# Autodesk Inventor assembly: ensamble
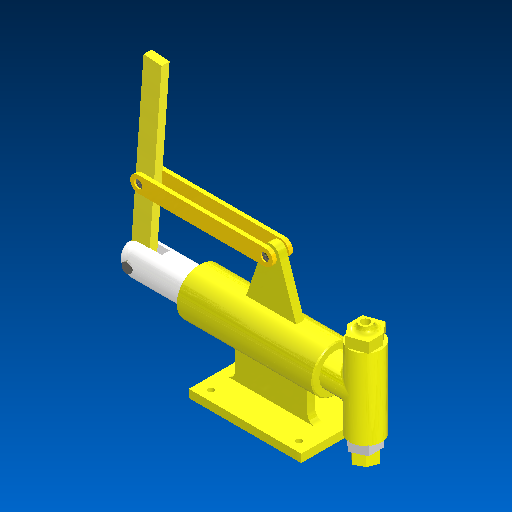
[picture p0: Inventor's stored thumbnail of the model, 512x512]
Saved by Autodesk Inventor 2025.2 (Build 292293000, 293)
## iProperties
Created: 2024-11-13
Part Number: ensamble
Document SubType Name: Assembly
Designer: Steven C
Author: Steven C
## Documents named in this file (12)
- C:\Users\Steven C\Desktop\8-807\ensamble.iam
- C:\Users\Steven C\Desktop\8-807\1 HUDSON-8-28A-TDR HAND PUMP BASE BODY.ipt
- C:\Users\Steven C\Desktop\8-807\1 -HUDSON-8-31B-TDR HAND PUMP PISTON.ipt
- C:\Users\Steven C\Desktop\8-807\1-HUDSON-8-29-TDR HAND PUMP BODY TOP OUTLET.ipt
- C:\Users\Steven C\Desktop\8-807\1-HUDSON-8-30-TDR HAND PUMP BODY BOTTOM INLET.ipt
- C:\Users\Steven C\Desktop\8-807\1-HUDSON-8-33-TDR HAND PUMP HANDLE.ipt
- C:\Users\Steven C\Desktop\8-807\2 HUDSON-8-31A-TDR HAND PUMP BALL VALVE.ipt
- C:\Users\Steven C\Desktop\8-807\2-HUDSON-8-32-TDR HAND PUMP LINK.ipt
- C:\Users\Steven C\Desktop\8-807\2-HUDSON-8-35-TDR HAND PUMP M8x5 PIPE NU.ipt
- C:\Users\Steven C\Documents\Inventor\Content Center Files\R2025\es-ES\BS 1804\BS 1804-2 - 4 x 10.ipt
- C:\Users\Steven C\Documents\Inventor\Content Center Files\R2025\es-ES\ISO 2338(5)\ISO 2338 - 5 h11 x 16 - CDIN EN.ipt
- C:\Users\Steven C\Desktop\8-807\1 HUDSON-8-28B-TDR HAND PUMP BASE BODY.ipt
## Components (14 placed, 11 different names)
1. 1 HUDSON-8-28A-TDR HAND PUMP BASE BODY:1 — Cilíndrica:1, Coincidencia:5, De rotación:1
2. 1 -HUDSON-8-31B-TDR HAND PUMP PISTON:1 — Coincidencia:5, Coincidencia:6, Coincidencia:7
3. 1-HUDSON-8-29-TDR HAND PUMP BODY TOP OUTLET:1 — De rotación:3, De rotación:4
4. 1-HUDSON-8-30-TDR HAND PUMP BODY BOTTOM INLET:1 — De rotación:2
5. 1-HUDSON-8-33-TDR HAND PUMP HANDLE:1 — Cilíndrica:2, Coincidencia:6, Cilíndrica:3
6. 2-HUDSON-8-31A-TDR HAND PUMP BALL VALVE:1 — Rígido:1
7. 2-HUDSON-8-35-TDR HAND PUMP M8x5 PIPE NU:1 — De rotación:4
8. 2-HUDSON-8-32-TDR HAND PUMP LINK:2 — Coincidencia:1, Coincidencia:4
9. BS 1804 : Pieza 2 4 x 10:1 — Cilíndrica:1, Coincidencia:1, Coincidencia:2, Coincidencia:3
10. 2-HUDSON-8-32-TDR HAND PUMP LINK:3 — Coincidencia:2, Coincidencia:3
11. BS 1804 : Pieza 2 4 x 10:2 — Coincidencia:4, Cilíndrica:2
12. DIN EN 22338 C - retirado 5 h11 x 16 - C:1 — Cilíndrica:3, Coincidencia:7
13. 1 HUDSON-8-28B-TDR HAND PUMP BASE BODY:2 — De rotación:1, Rígido:1, Rígido:2, De rotación:2, De rotación:3
14. 2-HUDSON-8-31A-TDR HAND PUMP BALL VALVE:2 — Rígido:2
## Relationships (16: Mate 7, RevoluteJoint 4, CylindricalJoint 3, WeldJoint 2)
- Cilíndrica:1 [CylindricalJoint]: 1 HUDSON-8-28A-TDR HAND PUMP BASE BODY:1 ↔ BS 1804 : Pieza 2 4 x 10:1
- Coincidencia:1 [Mate]: 2-HUDSON-8-32-TDR HAND PUMP LINK:2 ↔ BS 1804 : Pieza 2 4 x 10:1
- Coincidencia:2 [Mate]: BS 1804 : Pieza 2 4 x 10:1 ↔ 2-HUDSON-8-32-TDR HAND PUMP LINK:3
- Coincidencia:3 [Mate]: BS 1804 : Pieza 2 4 x 10:1 ↔ 2-HUDSON-8-32-TDR HAND PUMP LINK:3
- Coincidencia:4 [Mate]: 2-HUDSON-8-32-TDR HAND PUMP LINK:2 ↔ BS 1804 : Pieza 2 4 x 10:2
- Coincidencia:5 [Mate]: 1 HUDSON-8-28A-TDR HAND PUMP BASE BODY:1 ↔ 1 -HUDSON-8-31B-TDR HAND PUMP PISTON:1
- Cilíndrica:2 [CylindricalJoint]: 1-HUDSON-8-33-TDR HAND PUMP HANDLE:1 ↔ BS 1804 : Pieza 2 4 x 10:2
- Coincidencia:6 [Mate]: 1 -HUDSON-8-31B-TDR HAND PUMP PISTON:1 ↔ 1-HUDSON-8-33-TDR HAND PUMP HANDLE:1
- Cilíndrica:3 [CylindricalJoint]: 1-HUDSON-8-33-TDR HAND PUMP HANDLE:1 ↔ DIN EN 22338 C - retirado 5 h11 x 16 - C:1
- Coincidencia:7 [Mate]: 1 -HUDSON-8-31B-TDR HAND PUMP PISTON:1 ↔ DIN EN 22338 C - retirado 5 h11 x 16 - C:1
- De rotación:1 [RevoluteJoint]: 1 HUDSON-8-28A-TDR HAND PUMP BASE BODY:1 ↔ 1 HUDSON-8-28B-TDR HAND PUMP BASE BODY:2
- Rígido:1 [WeldJoint]: 2-HUDSON-8-31A-TDR HAND PUMP BALL VALVE:1 ↔ 1 HUDSON-8-28B-TDR HAND PUMP BASE BODY:2
- Rígido:2 [WeldJoint]: 1 HUDSON-8-28B-TDR HAND PUMP BASE BODY:2 ↔ 2-HUDSON-8-31A-TDR HAND PUMP BALL VALVE:2
- De rotación:2 [RevoluteJoint]: 1-HUDSON-8-30-TDR HAND PUMP BODY BOTTOM INLET:1 ↔ 1 HUDSON-8-28B-TDR HAND PUMP BASE BODY:2
- De rotación:3 [RevoluteJoint]: 1-HUDSON-8-29-TDR HAND PUMP BODY TOP OUTLET:1 ↔ 1 HUDSON-8-28B-TDR HAND PUMP BASE BODY:2
- De rotación:4 [RevoluteJoint]: 1-HUDSON-8-29-TDR HAND PUMP BODY TOP OUTLET:1 ↔ 2-HUDSON-8-35-TDR HAND PUMP M8x5 PIPE NU:1
